# Autodesk Inventor assembly: X Carriage-Unit
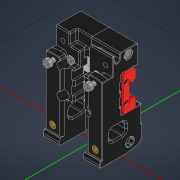
[picture p0: Inventor's stored thumbnail of the model, 180x180]
Saved by Autodesk Inventor 2022.2 (Build 262287010, 287A)
## iProperties
Created: 2022-03-15
Part Number: X Carriage-Unit
Document SubType Name: Assembly
Designer: sleib
Author: sleib
## Documents named in this file (10)
- C:\Users\sleib\Projekte\Voron-2\CAD\Inventor\X Carriage-Unit.iam
- C:\Users\sleib\Projekte\Voron-2\CAD\Inventor\X Carriage Left.ipt
- C:\Users\sleib\Projekte\Voron-2\CAD\Inventor\X Carriage Right.ipt
- C:\Users\sleib\Projekte\Voron-2\CAD\Inventor\M3 Hexnut.ipt
- C:\Users\sleib\Projekte\Voron-2\CAD\Inventor\M3x40 SHCS.ipt
- C:\Users\sleib\Projekte\Voron-2\CAD\Inventor\M3x30 SHCS.ipt
- C:\Users\sleib\Projekte\Voron-2\CAD\Inventor\M3 Threaded Insert.ipt
- C:\Users\sleib\Projekte\Voron-2\CAD\Inventor\MGN12H Carriage.iam
- C:\Users\sleib\Projekte\Voron-2\CAD\Inventor\M3x12 SHCS.ipt
- C:\Users\sleib\Projekte\Voron-2\CAD\Inventor\M3x8 SHCS.ipt
## Components (15 placed, 9 different names)
1. X Carriage Left:1 — Fluchtend:1, Fluchtend:2, Passend:5, Passend:10, Passend:12, Fluchtend:5, Passend:19, Passend:20, Passend:27, Passend:29, Passend:30
2. X Carriage Right:1 — Passend:1, Fluchtend:3, Passend:2, Passend:3, Passend:4, Winkel:1, Winkel:2, Passend:6, Passend:7, Passend:13, Fluchtend:4, Passend:18, Passend:21, Passend:26, Passend:28, Passend:31
3. M3 Hexnut:1 — Passend:2, Winkel:1, Passend:6, Passend:8
4. M3 Hexnut:2 — Passend:3, Winkel:2, Passend:7
5. M3x30 SHCS:1
6. M3x40 SHCS:2 — Passend:8, Passend:10
7. M3 Threaded Insert:1 — Passend:12, Fluchtend:5
8. M3 Threaded Insert:2 — Passend:13, Fluchtend:4
9. MGN12H Carriage:1 [sub-assembly] — Passend:22, Passend:23, Passend:24, Passend:25, Passend:26, Passend:27
10. M3x8 SHCS:1 — Passend:19, Passend:22
11. M3x8 SHCS:2 — Passend:20, Passend:25
12. M3x8 SHCS:3 — Passend:18, Passend:23
13. M3x8 SHCS:4 — Passend:21, Passend:24
14. M3x12 SHCS:1 — Passend:28, Passend:31
15. M3x12 SHCS:2 — Passend:29, Passend:30
## Relationships (38: Mate 31, Flush 5, Angle 2)
- Fluchtend:1 [Flush]: X Carriage Left:1
- Passend:1 [Mate]: X Carriage Right:1
- Fluchtend:2 [Flush]: X Carriage Left:1
- Fluchtend:3 [Flush]: X Carriage Right:1
- Passend:2 [Mate]: X Carriage Right:1 ↔ M3 Hexnut:1
- Passend:3 [Mate]: X Carriage Right:1 ↔ M3 Hexnut:2
- Passend:4 [Mate] (10 mm): X Carriage Right:1
- Passend:5 [Mate] (10 mm): X Carriage Left:1
- Winkel:1 [Angle] (0 deg): X Carriage Right:1 ↔ M3 Hexnut:1
- Winkel:2 [Angle] (0 deg): X Carriage Right:1 ↔ M3 Hexnut:2
- Passend:6 [Mate]: X Carriage Right:1 ↔ M3 Hexnut:1
- Passend:7 [Mate]: X Carriage Right:1 ↔ M3 Hexnut:2
- Passend:8 [Mate]: M3 Hexnut:1 ↔ M3x40 SHCS:2
- [Mate]: M3 Hexnut:2 ↔ M3x30 SHCS:1
- Passend:10 [Mate]: X Carriage Left:1 ↔ M3x40 SHCS:2
- [Mate]: X Carriage Left:1 ↔ M3x30 SHCS:1
- Passend:12 [Mate]: X Carriage Left:1 ↔ M3 Threaded Insert:1
- Passend:13 [Mate]: X Carriage Right:1 ↔ M3 Threaded Insert:2
- Fluchtend:4 [Flush]: X Carriage Right:1 ↔ M3 Threaded Insert:2
- Fluchtend:5 [Flush]: X Carriage Left:1 ↔ M3 Threaded Insert:1
- [Mate]: X Carriage Left:1 ↔ M3x8 SHCS:1
- [Mate]: X Carriage Left:1 ↔ M3x8 SHCS:2
- [Mate]: X Carriage Right:1 ↔ M3x8 SHCS:3
- [Mate]: X Carriage Right:1 ↔ M3x8 SHCS:4
- Passend:18 [Mate]: X Carriage Right:1 ↔ M3x8 SHCS:3
- Passend:19 [Mate]: X Carriage Left:1 ↔ M3x8 SHCS:1
- Passend:20 [Mate]: X Carriage Left:1 ↔ M3x8 SHCS:2
- Passend:21 [Mate]: X Carriage Right:1 ↔ M3x8 SHCS:4
- Passend:22 [Mate]: MGN12H Carriage:1 ↔ M3x8 SHCS:1
- Passend:23 [Mate]: MGN12H Carriage:1 ↔ M3x8 SHCS:3
- Passend:24 [Mate]: MGN12H Carriage:1 ↔ M3x8 SHCS:4
- Passend:25 [Mate]: MGN12H Carriage:1 ↔ M3x8 SHCS:2
- Passend:26 [Mate]: X Carriage Right:1 ↔ MGN12H Carriage:1
- Passend:27 [Mate]: X Carriage Left:1 ↔ MGN12H Carriage:1
- Passend:28 [Mate]: X Carriage Right:1 ↔ M3x12 SHCS:1
- Passend:29 [Mate]: X Carriage Left:1 ↔ M3x12 SHCS:2
- Passend:30 [Mate] (3 mm): X Carriage Left:1 ↔ M3x12 SHCS:2
- Passend:31 [Mate] (3 mm): X Carriage Right:1 ↔ M3x12 SHCS:1
